# Autodesk Inventor assembly: treadle
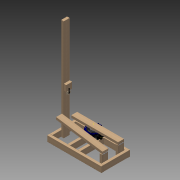
[picture p0: Inventor's stored thumbnail of the model, 180x180]
Saved by Autodesk Inventor 2014 (Build 180170000, 170)
## iProperties
Created: 2013-10-13
Part Number: treadle
Document SubType Name: Assembly
Designer: david
Author: david
## Documents named in this file (11)
- C:\Users\david\Documents\GitHub\CAD\treadle.iam
- C:\Users\david\Documents\GitHub\CAD\2x4x14.ipt
- C:\Users\david\Documents\GitHub\CAD\2x4x32.ipt
- C:\Users\david\Documents\GitHub\CAD\2x4x7.75.ipt
- C:\Users\david\Documents\GitHub\CAD\hinge 3 holes.ipt
- C:\Users\david\Documents\GitHub\CAD\hinge 2 holes.ipt
- C:\Users\david\Documents\GitHub\CAD\2x4x27.75.ipt
- C:\Users\david\Documents\GitHub\CAD\2x4x60.ipt
- C:\Users\david\Documents\GitHub\CAD\2x4x3.5.ipt
- C:\Users\david\Documents\GitHub\CAD\Pulley.iam
- C:\Users\david\Documents\GitHub\CAD\amazon_universal.iam
## Components (18 placed, 10 different names)
1. 2x4x14:2 — Mate:2, Flush:3, Flush:4, Mate:17
2. 2x4x14:4 — Mate:1, Flush:1, Flush:2, Mate:3, Flush:5, Mate:7, Flush:10, Flush:11, Mate:8, Flush:12, Flush:17, Mate:20, Mate:22
3. 2x4x32:1 — Mate:1, Flush:1, Flush:2, Mate:2, Flush:3, Flush:4, Mate:4, Mate:18
4. 2x4x7.75:1 — Mate:3, Flush:5, Mate:4, Mate:5, Flush:6, Flush:7
5. hinge 3 holes:1 — Mate:5, Flush:6, Flush:7, Rotational:1
6. hinge 2 holes:1 — Rotational:1, Mate:6, Flush:8, Flush:9
7. 2x4x27.75:1 — Mate:6, Flush:8, Flush:9
8. 2x4x32:2 — Mate:7, Flush:10, Flush:11, Mate:9, Mate:19, Flush:21, Mate:21, Flush:22
9. 2x4x7.75:2 — Mate:8, Mate:9, Flush:12, Mate:10, Flush:13, Flush:14, Flush:16
10. hinge 3 holes:2 — Mate:10, Flush:13, Flush:14, Rotational:2
11. hinge 2 holes:2 — Rotational:2, Mate:11, Flush:15
12. 2x4x27.75:2 — Mate:11, Flush:15, Flush:16, Mate:24, Flush:23, Mate:25
13. 2x4x60:1 — Flush:17, Mate:14, Flush:18, Flush:19, Mate:17, Mate:18
14. 2x4x3.5:1 — Mate:14, Flush:18, Flush:19, Mate:15, Flush:20, Mate:16
15. Pulley:1 [sub-assembly] — Mate:15, Flush:20, Mate:16
16. 2x4x14:5 — Mate:21, Flush:22, Mate:22
17. 2x4x14:6 — Mate:19, Flush:21, Mate:20, Mate:23
18. amazon_universal:1 [sub-assembly] — Mate:23, Mate:24, Flush:23, Mate:25
## Relationships (48: Mate 23, Flush 23, RevoluteJoint 2)
- Mate:1: 2x4x14:4 ↔ 2x4x32:1
- Flush:1: 2x4x14:4 ↔ 2x4x32:1
- Flush:2: 2x4x14:4 ↔ 2x4x32:1
- Mate:2: 2x4x14:2 ↔ 2x4x32:1
- Flush:3: 2x4x14:2 ↔ 2x4x32:1
- Flush:4: 2x4x14:2 ↔ 2x4x32:1
- Mate:3: 2x4x14:4 ↔ 2x4x7.75:1
- Flush:5: 2x4x14:4 ↔ 2x4x7.75:1
- Mate:4 (12.7 mm): 2x4x32:1 ↔ 2x4x7.75:1
- Mate:5: 2x4x7.75:1 ↔ hinge 3 holes:1
- Flush:6: 2x4x7.75:1 ↔ hinge 3 holes:1
- Flush:7 (-6.35 mm): 2x4x7.75:1 ↔ hinge 3 holes:1
- Rotational:1 [RevoluteJoint]: hinge 3 holes:1 ↔ hinge 2 holes:1
- Mate:6: hinge 2 holes:1 ↔ 2x4x27.75:1
- Flush:8: hinge 2 holes:1 ↔ 2x4x27.75:1
- Flush:9 (-6.35 mm): hinge 2 holes:1 ↔ 2x4x27.75:1
- Mate:7: 2x4x14:4 ↔ 2x4x32:2
- Flush:10: 2x4x14:4 ↔ 2x4x32:2
- Flush:11: 2x4x14:4 ↔ 2x4x32:2
- Mate:8: 2x4x14:4 ↔ 2x4x7.75:2
- Mate:9 (12.7 mm): 2x4x32:2 ↔ 2x4x7.75:2
- Flush:12: 2x4x14:4 ↔ 2x4x7.75:2
- Mate:10: 2x4x7.75:2 ↔ hinge 3 holes:2
- Flush:13: 2x4x7.75:2 ↔ hinge 3 holes:2
- Flush:14 (-6.35 mm): 2x4x7.75:2 ↔ hinge 3 holes:2
- Rotational:2 [RevoluteJoint]: hinge 3 holes:2 ↔ hinge 2 holes:2
- Mate:11: hinge 2 holes:2 ↔ 2x4x27.75:2
- Flush:15: hinge 2 holes:2 ↔ 2x4x27.75:2
- Flush:16: 2x4x7.75:2 ↔ 2x4x27.75:2
- Flush:17: 2x4x14:4 ↔ 2x4x60:1
- Mate:14: 2x4x60:1 ↔ 2x4x3.5:1
- Flush:18: 2x4x60:1 ↔ 2x4x3.5:1
- Flush:19 (-622.3 mm): 2x4x60:1 ↔ 2x4x3.5:1
- Mate:15: 2x4x3.5:1 ↔ Pulley:1
- Flush:20: 2x4x3.5:1 ↔ Pulley:1
- Mate:16 (12.7 mm): 2x4x3.5:1 ↔ Pulley:1
- Mate:17: 2x4x14:2 ↔ 2x4x60:1
- Mate:18 (133.35 mm): 2x4x32:1 ↔ 2x4x60:1
- Mate:19: 2x4x32:2 ↔ 2x4x14:6
- Flush:21: 2x4x32:2 ↔ 2x4x14:6
- Mate:20 (317.5 mm): 2x4x14:4 ↔ 2x4x14:6
- Mate:21: 2x4x32:2 ↔ 2x4x14:5
- Flush:22: 2x4x32:2 ↔ 2x4x14:5
- Mate:22 (469.9 mm): 2x4x14:4 ↔ 2x4x14:5
- Mate:23: 2x4x14:6 ↔ amazon_universal:1
- Mate:24: 2x4x27.75:2 ↔ amazon_universal:1
- Flush:23 (406.4 mm): 2x4x27.75:2 ↔ amazon_universal:1
- Mate:25: 2x4x27.75:2 ↔ amazon_universal:1
